# Autodesk Inventor assembly: GBK-ASY щит стеновой 1.1
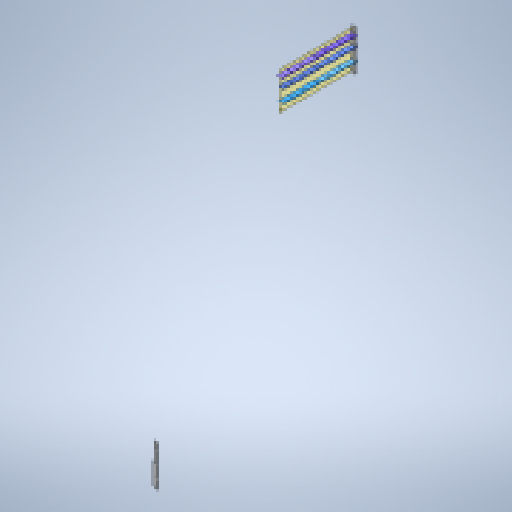
[picture p0: Inventor's stored thumbnail of the model, 512x512]
Saved by Autodesk Inventor 2026.2 (Build 302298000, 298)
## iProperties
Created: 2026-05-07
Part Number: GBK-ASY щит стеновой 1.1
Document SubType Name: Assembly
Designer: admin
Mass: 245734 g
Surface Area: 167509 cm^2
Volume: 31303.7 cm^3
Density: 7.85 g/cm^3
Author: admin
## Documents named in this file (7)
- C:\Users\admin\Documents\Inventor\GBK-Gubkinskiy\Assembly shield 1.iam
- C:\Users\admin\Documents\Inventor\GBK-Gubkinskiy\Part111.ipt
- C:\Users\admin\Documents\Inventor\GBK-Gubkinskiy\stringer 1.ipt
- C:\Users\admin\Documents\Inventor\GBK-Gubkinskiy\stringer 1.2.ipt
- C:\Users\admin\Documents\Inventor\GBK-Gubkinskiy\Part2.ipt
- C:\Users\admin\Documents\Inventor\GBK-Gubkinskiy\stringer 1.3.ipt
- C:\Users\admin\Documents\Inventor\GBK-Gubkinskiy\Part2_CPY1.ipt
## Components (9 placed, 6 different names)
1. Part111:1
2. stringer 1:1
3. stringer 1.2:1
4. stringer 1:2
5. Part2:1
6. stringer 1.3:1
7. stringer 1.2:2
8. stringer 1.3:2
9. Part2_CPY1:1
## Relationships (3: WeldJoint 3)
- [WeldJoint]: stringer 1:1 ↔ stringer 1:2
- [WeldJoint]: stringer 1.2:1 ↔ stringer 1.2:2
- [WeldJoint]: stringer 1.3:1 ↔ stringer 1.3:2
